# Autodesk Inventor assembly: 42146-34
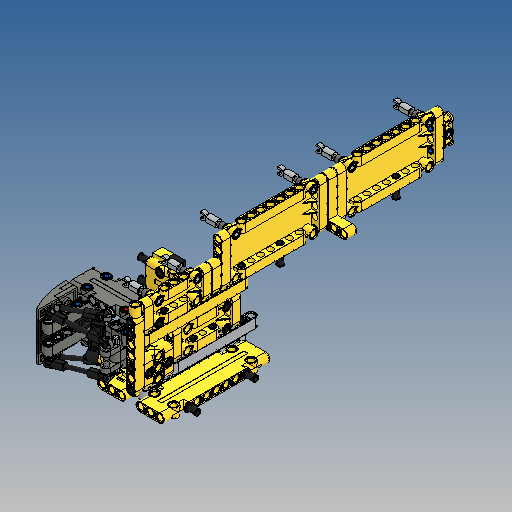
[picture p0: Inventor's stored thumbnail of the model, 512x512]
Saved by Autodesk Inventor 2025 (Build 290162010, 162A)
## iProperties
Created: 2024-12-06
Part Number: 42146-34
Material: Generisch
Document SubType Name: Assembly
Designer: hp.muther
Author: hp.muther
## Documents named in this file (48)
- D:\Inventor\Projekte\Muther\LEGO Technic\LEGO Technik - Raupenkran LR 13000 (42146)\42146-34.iam
- D:\Inventor\Projekte\Muther\LEGO Technic\LEGO Pieces\Paneelen\18945-Yellow.ipt
- D:\Inventor\Projekte\Muther\LEGO Technic\LEGO Pieces\Lochbalken\73507-LtBluishGray.ipt
- D:\Inventor\Projekte\Muther\LEGO Technic\LEGO Pieces\Paneelen\15458-Yellow.ipt
- D:\Inventor\Projekte\Muther\LEGO Technic\LEGO Pieces\Pin's\6558-Blue.ipt
- D:\Inventor\Projekte\Muther\LEGO Technic\LEGO Pieces\Pin's\2780-Black.ipt
- D:\Inventor\Projekte\Muther\LEGO Technic\LEGO Pieces\Pin's\32054-LtBluishGray.ipt
- D:\Inventor\Projekte\Muther\LEGO Technic\LEGO Pieces\Pin's\43093-Blue.ipt
- D:\Inventor\Projekte\Muther\LEGO Technic\LEGO Pieces\Pin's\4274-LtBluishGray.ipt
- D:\Inventor\Projekte\Muther\LEGO Technic\LEGO Pieces\Verbindungselemente\32184-Yellow.ipt
- D:\Inventor\Projekte\Muther\LEGO Technic\LEGO Pieces\Verbindungselemente\39793-Yellow.ipt
- D:\Inventor\Projekte\Muther\LEGO Technic\LEGO Pieces\Winkel\32526-Yellow.ipt
- D:\Inventor\Projekte\Muther\LEGO Technic\LEGO Pieces\Lochbalken\32523-Yellow.ipt
- D:\Inventor\Projekte\Muther\LEGO Technic\LEGO Pieces\Lochbalken\32525-Yellow.ipt
- D:\Inventor\Projekte\Muther\LEGO Technic\LEGO Pieces\Lochbalken\32524-Yellow.ipt
- D:\Inventor\Projekte\Muther\LEGO Technic\LEGO Pieces\Lochbalken\40490-LtBluishGray.ipt
- D:\Inventor\Projekte\Muther\LEGO Technic\LEGO Pieces\Paneelen\64782-Yellow.ipt
- D:\Inventor\Projekte\Muther\LEGO Technic\LEGO Pieces\Paneelen\71709-Yellow.ipt
- D:\Inventor\Projekte\Muther\LEGO Technic\LEGO Pieces\Verbindungselemente\15100-Yellow.ipt
- D:\Inventor\Projekte\Muther\LEGO Technic\LEGO Pieces\Achsen\78258-DarkStoneGrey.ipt
- D:\Inventor\Projekte\Muther\LEGO Technic\LEGO Pieces\Diverses\44873-LtBluishGray.ipt
- D:\Inventor\Projekte\Muther\LEGO Technic\LEGO Pieces\Steine\32000-Black.ipt
- D:\Inventor\Projekte\Muther\LEGO Technic\LEGO Pieces\Steine\3894-Yellow.ipt
- D:\Inventor\Projekte\Muther\LEGO Technic\LEGO Pieces\Lochbalken\32524-DkBluishGray.ipt
- D:\Inventor\Projekte\Muther\LEGO Technic\LEGO Pieces\Rund\18654-DkBluishGray.ipt
- D:\Inventor\Projekte\Muther\LEGO Technic\LEGO Pieces\Winkel\32140-DkBluishGray.ipt
- D:\Inventor\Projekte\Muther\LEGO Technic\LEGO Pieces\Paneelen\71709-DkBluishGray.ipt
- D:\Inventor\Projekte\Muther\LEGO Technic\LEGO Pieces\Winkel\32056-DkBluishGray.ipt
- D:\Inventor\Projekte\Muther\LEGO Technic\LEGO Pieces\Pin's\11214-Red.ipt
- D:\Inventor\Projekte\Muther\LEGO Technic\LEGO Pieces\Platten, Kacheln\18677-Black.ipt
- D:\Inventor\Projekte\Muther\LEGO Technic\LEGO Technik - Raupenkran LR 13000 (42146)\42146_63864_1.ipt
- D:\Inventor\Projekte\Muther\LEGO Technic\LEGO Pieces\Lochbalken\60483-DkBluishGray.ipt
- D:\Inventor\Projekte\Muther\LEGO Technic\LEGO Pieces\Lochbalken schmal\41677-DKBluishGray.ipt
- D:\Inventor\Projekte\Muther\LEGO Technic\LEGO Pieces\Achsen\4519-LtBluishGray.ipt
- D:\Inventor\Projekte\Muther\LEGO Technic\LEGO Pieces\Diverses\48729-DkBluishGray.ipt
- D:\Inventor\Projekte\Muther\LEGO Technic\LEGO Pieces\Achsen\87994-Black.ipt
- D:\Inventor\Projekte\Muther\LEGO Technic\LEGO Pieces\Diverses\23443-Black.ipt
- D:\Inventor\Projekte\Muther\LEGO Technic\LEGO Pieces\Steine rund\98138-TransOrange.ipt
- D:\Inventor\Projekte\Muther\LEGO Technic\LEGO Pieces\Platten, Kacheln\63864-DkBluishGray.ipt
- D:\Inventor\Projekte\Muther\LEGO Technic\LEGO Pieces\Platten, Kacheln\3623-DkBluishGray.ipt
- D:\Inventor\Projekte\Muther\LEGO Technic\LEGO Pieces\Platten, Kacheln\3021-DkBluishGray.ipt
- D:\Inventor\Projekte\Muther\LEGO Technic\LEGO Pieces\Platten, Kacheln\3022-DkBluishGray.ipt
- D:\Inventor\Projekte\Muther\LEGO Technic\LEGO Pieces\Steine schräg\11153-Black.ipt
- D:\Inventor\Projekte\Muther\LEGO Technic\LEGO Pieces\Platten, Kacheln\11212-DkBluishGray.ipt
- D:\Inventor\Projekte\Muther\LEGO Technic\LEGO Pieces\Steine schräg\11153-DkBluishGray.ipt
- D:\Inventor\Projekte\Muther\LEGO Technic\LEGO Pieces\Platten, Kacheln\3070-DkBluishGray.ipt
- D:\Inventor\Projekte\Muther\LEGO Technic\LEGO Pieces\Platten, Kacheln\3024-DkBluishGray.ipt
- D:\Inventor\Projekte\Muther\LEGO Technic\LEGO Pieces\Platten, Kacheln\93606-Black.ipt
## Components (147 placed, 47 different names)
1. 18945-Yellow:1 — Einfügen:1, Einfügen:6, Passend:2
2. 73507-LtBluishGray:1 — Einfügen:2, Einfügen:3, Einfügen:6, Einfügen:7, Einfügen:45, Passend:12
3. 15458-Yellow:1 — Einfügen:4, Einfügen:5, Einfügen:7, Passend:1
4. 6558-Blue:1 — Einfügen:2
5. 6558-Blue:2 — Einfügen:3, Passend:1, Passend:2
6. 2780-Black:1 — Einfügen:4
7. 32054-LtBluishGray:1 — Einfügen:1
8. 2780-Black:2 — Einfügen:5
9. 43093-Blue:1 — Einfügen:8
10. 43093-Blue:2 — Einfügen:9, Passend:3
11. 6558-Blue:3 — Einfügen:11, Passend:4, Passend:5
12. 6558-Blue:4 — Einfügen:12
13. 2780-Black:3 — Einfügen:15, Passend:8
14. 6558-Blue:5 — Einfügen:16
15. 6558-Blue:6 — Einfügen:17, Passend:6, Passend:7
16. 2780-Black:4 — Einfügen:21
17. 2780-Black:5 — Einfügen:20
18. 2780-Black:6 — Einfügen:19
19. 2780-Black:7 — Einfügen:30
20. 2780-Black:8 — Einfügen:31, Passend:11
21. 2780-Black:9 — Einfügen:26, Passend:10
22. 2780-Black:12 — Einfügen:27, Passend:9
23. 2780-Black:13 — Einfügen:28
24. 2780-Black:14 — Einfügen:34, Passend:12
25. 2780-Black:15 — Einfügen:35
26. 2780-Black:16 — Einfügen:36
27. 2780-Black:17 — Einfügen:37
28. 4274-LtBluishGray:1 — Einfügen:46, Einfügen:48
29. 2780-Black:18 — Einfügen:40, Passend:78
30. 2780-Black:19 — Einfügen:41
31. 2780-Black:20 — Einfügen:42
32. 2780-Black:21 — Einfügen:43, Passend:21
33. 2780-Black:22 — Einfügen:44, Passend:79
34. 32184-Yellow:1 — Einfügen:8, Einfügen:9, Einfügen:10, Einfügen:66
35. 39793-Yellow:1 — Einfügen:30, Einfügen:31, Einfügen:32, Fluchtend:1, Einfügen:40, Einfügen:41, Passend:77
36. 32526-Yellow:1 — Einfügen:11, Einfügen:12, Einfügen:13, Einfügen:14
37. 32523-Yellow:1 — Einfügen:16, Einfügen:17, Einfügen:18, Einfügen:22
38. 32525-Yellow:1 — Einfügen:23, Passend:8, Einfügen:29, Passend:9
39. 32524-Yellow:1 — Einfügen:39, Passend:11
40. 40490-LtBluishGray:1 — Einfügen:33, Passend:10, Einfügen:34, Einfügen:35, Einfügen:45
41. 64782-Yellow:1 — Einfügen:10, Passend:3, Einfügen:13, Passend:4, Einfügen:37, Einfügen:64, Einfügen:65
42. 71709-Yellow:1 — Einfügen:19, Einfügen:20, Einfügen:21, Einfügen:22, Passend:7, Einfügen:23, Einfügen:38, Fluchtend:2, Einfügen:39, Einfügen:44, Einfügen:46, Einfügen:61
43. 15100-Yellow:1 — Einfügen:38, Fluchtend:2
44. 64782-Yellow:2 — Einfügen:14, Passend:5, Einfügen:18, Passend:6, Einfügen:15, Einfügen:36, Einfügen:62, Einfügen:63
45. 2780-Black:23
46. 2780-Black:24
47. 71709-Yellow:2 — Einfügen:26, Einfügen:27, Einfügen:28, Einfügen:29, Einfügen:32, Fluchtend:1, Einfügen:33, Einfügen:42, Einfügen:43, Einfügen:72
48. 44873-LtBluishGray:1 — Einfügen:47, Passend:13
49. 78258-DarkStoneGrey:1 — Einfügen:47, Einfügen:48
50. 4274-LtBluishGray:2 — Einfügen:61
51. 44873-LtBluishGray:2 — Passend:13
52. 78258-DarkStoneGrey:2
53. 4274-LtBluishGray:3 — Einfügen:62
54. 44873-LtBluishGray:3 — Passend:14
55. 78258-DarkStoneGrey:3
56. 4274-LtBluishGray:4 — Einfügen:63
57. 44873-LtBluishGray:4 — Passend:14, Passend:15
58. 78258-DarkStoneGrey:4
59. 4274-LtBluishGray:5 — Einfügen:66
60. 44873-LtBluishGray:5 — Winkel:1
61. 78258-DarkStoneGrey:5
62. 4274-LtBluishGray:6 — Einfügen:65
63. 44873-LtBluishGray:6 — Passend:16, Winkel:1
64. 78258-DarkStoneGrey:6
65. 4274-LtBluishGray:7 — Einfügen:64
66. 44873-LtBluishGray:7 — Passend:15, Passend:16
67. 78258-DarkStoneGrey:7
68. 2780-Black:25 — Einfügen:67, Passend:20
69. 2780-Black:26 — Einfügen:68
70. 71709-Yellow:3 — Einfügen:67, Einfügen:68, Einfügen:69, Einfügen:70, Einfügen:71, Einfügen:72, Passend:21
71. 2780-Black:27 — Einfügen:70
72. 2780-Black:28 — Einfügen:69
73. 32000-Black:1 — Passend:18, Fluchtend:5, Passend:19, Passend:20
74. 32000-Black:2 — Passend:17, Fluchtend:3, Fluchtend:4, Passend:19, Einfügen:71
75. 3894-Yellow:1 — Passend:17, Passend:18, Fluchtend:3, Fluchtend:4, Fluchtend:5
76. 32524-DkBluishGray:1 — Einfügen:73, Einfügen:74, Einfügen:77, Einfügen:78, Einfügen:79, Einfügen:80, Einfügen:81, Einfügen:82, Einfügen:85
77. 32000-Black:3 — Einfügen:81, Passend:75
78. 32000-Black:4 — Einfügen:82, Einfügen:83, Fluchtend:18
79. 4274-LtBluishGray:8 — Einfügen:73, Einfügen:108
80. 4274-LtBluishGray:9 — Einfügen:74, Einfügen:109
81. 6558-Blue:7 — Einfügen:77
82. 6558-Blue:8 — Einfügen:80, Passend:24
83. 6558-Blue:9 — Einfügen:79, Passend:23
84. 6558-Blue:10 — Einfügen:78
85. 32524-DkBluishGray:2 — Einfügen:83, Passend:23, Einfügen:103, Einfügen:104, Einfügen:107
86. 4274-LtBluishGray:10 — Einfügen:111
87. 4274-LtBluishGray:11 — Einfügen:110
88. 4274-LtBluishGray:12 — Einfügen:84, Einfügen:113
89. 6558-Blue:11 — Einfügen:87, Passend:31
90. 43093-Blue:3 — Einfügen:86, Einfügen:88
91. 18654-DkBluishGray:1 — Einfügen:89
92. 32140-DkBluishGray:1 — Einfügen:88, Passend:25, Einfügen:89, Einfügen:87, Einfügen:93, Passend:27, Einfügen:100
93. 71709-DkBluishGray:1 — Einfügen:84, Einfügen:85, Passend:24, Einfügen:86, Passend:25, Passend:76, Passend:79
94. 32056-DkBluishGray:1 — Einfügen:90, Passend:26, Einfügen:92, Einfügen:94, Winkel:2, Winkel:3
95. 32056-DkBluishGray:2 — Einfügen:90, Passend:26, Einfügen:91, Passend:27
96. 43093-Blue:4 — Einfügen:92
97. 11214-Red:1 — Einfügen:91, Einfügen:93
98. 15100-Yellow:2 — Einfügen:94, Einfügen:95, Winkel:2
99. 18677-Black:1 — Passend:28, Fluchtend:6, Fluchtend:7, Einfügen:95
100. 42146_63864_1:1 — Passend:28, Fluchtend:6, Fluchtend:7
101. 6558-Blue:12 — Einfügen:99
102. 60483-DkBluishGray:1 — Einfügen:96, Einfügen:97, Einfügen:98, Einfügen:99, Einfügen:100, Winkel:3, Einfügen:101
103. 41677-DKBluishGray:1 — Einfügen:97, Passend:29, Einfügen:114
104. 41677-DKBluishGray:2 — Einfügen:98, Passend:30, Einfügen:115
105. 4519-LtBluishGray:1 — Einfügen:96, Passend:29, Passend:30
106. 32140-DkBluishGray:2 — Einfügen:101, Passend:31, Einfügen:102, Einfügen:106
107. 43093-Blue:5 — Einfügen:102
108. 2780-Black:29 — Einfügen:103
109. 2780-Black:30 — Einfügen:104
110. 71709-DkBluishGray:2 — Einfügen:105, Einfügen:107, Passend:32, Passend:77, Passend:78
111. 4274-LtBluishGray:13 — Einfügen:105, Einfügen:112
112. 2780-Black:31 — Einfügen:106, Passend:32
113. 48729-DkBluishGray:1 — Einfügen:108, Passend:35, Passend:36
114. 48729-DkBluishGray:2 — Einfügen:109, Einfügen:125
115. 48729-DkBluishGray:3 — Einfügen:113, Einfügen:120
116. 48729-DkBluishGray:4 — Einfügen:115, Einfügen:123
117. 48729-DkBluishGray:5 — Einfügen:110, Einfügen:124
118. 48729-DkBluishGray:6 — Einfügen:112, Einfügen:121
119. 48729-DkBluishGray:7 — Einfügen:111, Passend:37, Passend:38
120. 48729-DkBluishGray:8 — Einfügen:114, Einfügen:122
121. 87994-Black:1 — Einfügen:116, Passend:35, Passend:36
122. 23443-Black:1 — Einfügen:116, Einfügen:120
123. 87994-Black:2 — Passend:33
124. 23443-Black:2 — Einfügen:122
125. 23443-Black:3 — Passend:33, Einfügen:125
126. 87994-Black:3
127. 23443-Black:4 — Einfügen:123
128. 23443-Black:5 — Einfügen:124
129. 87994-Black:4 — Passend:37, Passend:38
130. 23443-Black:6 — Einfügen:121
131. 98138-TransOrange:1 — Einfügen:126
132. 63864-DkBluishGray:1 — Passend:47, Fluchtend:12, Fluchtend:13, Passend:49, Passend:53, Passend:54, Fluchtend:14, Passend:67, Passend:71, Passend:72
133. 63864-DkBluishGray:2 — Passend:57, Passend:58, Fluchtend:15, Passend:73
134. 3623-DkBluishGray:1 — Passend:39, Fluchtend:8, Fluchtend:9, Passend:41, Fluchtend:13
135. 3021-DkBluishGray:1 — Passend:42, Passend:43, Passend:45, Fluchtend:11, Passend:46, Passend:59
136. 3022-DkBluishGray:1 — Passend:44, Passend:45, Fluchtend:11, Passend:60
137. 11153-Black:1 — Passend:64, Passend:69, Passend:70, Passend:73
138. 11212-DkBluishGray:1 — Passend:39, Fluchtend:8, Fluchtend:9, Passend:40, Fluchtend:10, Passend:43, Passend:46, Passend:75, Passend:76, Fluchtend:18
139. 11153-DkBluishGray:1 — Passend:65, Passend:70, Passend:74
140. 11153-DkBluishGray:2 — Passend:66, Passend:67, Passend:68, Passend:71
141. 3070-DkBluishGray:1 — Passend:52, Passend:53, Passend:55, Passend:58, Fluchtend:15
142. 3070-DkBluishGray:2 — Passend:50, Passend:51, Passend:54, Passend:56, Fluchtend:14
143. 3024-DkBluishGray:1 — Passend:48, Passend:49, Passend:55, Passend:56, Einfügen:126
144. 93606-Black:1 — Passend:63, Passend:68, Passend:69, Passend:72
145. 11212-DkBluishGray:2 — Passend:40, Passend:41, Fluchtend:10, Passend:47, Fluchtend:12, Passend:48, Passend:50, Passend:42, Passend:51, Passend:52, Passend:57, Passend:61, Passend:62, Fluchtend:16, Fluchtend:17, Passend:44, Passend:63, Passend:64
146. 3024-DkBluishGray:2 — Passend:59, Passend:62, Fluchtend:16, Passend:66
147. 3024-DkBluishGray:3 — Passend:60, Passend:61, Fluchtend:17, Passend:65, Passend:74
## Relationships (226: Insert 126, Mate 79, Flush 18, Angle 3)
- Winkel:2 [Angle] (20 deg): 32056-DkBluishGray:1 ↔ 15100-Yellow:2
- Einfügen:1 [Insert]: 18945-Yellow:1 ↔ 32054-LtBluishGray:1
- Einfügen:2 [Insert]: 73507-LtBluishGray:1 ↔ 6558-Blue:1
- Einfügen:3 [Insert]: 73507-LtBluishGray:1 ↔ 6558-Blue:2
- Einfügen:4 [Insert]: 15458-Yellow:1 ↔ 2780-Black:1
- Einfügen:5 [Insert]: 15458-Yellow:1 ↔ 2780-Black:2
- Einfügen:6 [Insert]: 18945-Yellow:1 ↔ 73507-LtBluishGray:1
- Einfügen:7 [Insert]: 73507-LtBluishGray:1 ↔ 15458-Yellow:1
- Passend:1 [Mate]: 15458-Yellow:1 ↔ 6558-Blue:2
- Passend:2 [Mate]: 18945-Yellow:1 ↔ 6558-Blue:2
- Einfügen:8 [Insert]: 43093-Blue:1 ↔ 32184-Yellow:1
- Einfügen:9 [Insert]: 43093-Blue:2 ↔ 32184-Yellow:1
- Einfügen:10 [Insert]: 32184-Yellow:1 ↔ 64782-Yellow:1
- Passend:3 [Mate]: 43093-Blue:2 ↔ 64782-Yellow:1
- Einfügen:11 [Insert]: 6558-Blue:3 ↔ 32526-Yellow:1
- Einfügen:12 [Insert]: 6558-Blue:4 ↔ 32526-Yellow:1
- Einfügen:13 [Insert]: 32526-Yellow:1 ↔ 64782-Yellow:1
- Passend:4 [Mate]: 6558-Blue:3 ↔ 64782-Yellow:1
- Einfügen:14 [Insert]: 32526-Yellow:1 ↔ 64782-Yellow:2
- Passend:5 [Mate]: 6558-Blue:3 ↔ 64782-Yellow:2
- Einfügen:15 [Insert]: 2780-Black:3 ↔ 64782-Yellow:2
- Einfügen:16 [Insert]: 6558-Blue:5 ↔ 32523-Yellow:1
- Einfügen:17 [Insert]: 6558-Blue:6 ↔ 32523-Yellow:1
- Einfügen:18 [Insert]: 32523-Yellow:1 ↔ 64782-Yellow:2
- Passend:6 [Mate]: 6558-Blue:6 ↔ 64782-Yellow:2
- Einfügen:19 [Insert]: 2780-Black:6 ↔ 71709-Yellow:1
- Einfügen:20 [Insert]: 2780-Black:5 ↔ 71709-Yellow:1
- Einfügen:21 [Insert]: 2780-Black:4 ↔ 71709-Yellow:1
- Einfügen:22 [Insert]: 32523-Yellow:1 ↔ 71709-Yellow:1
- Passend:7 [Mate]: 6558-Blue:6 ↔ 71709-Yellow:1
- Einfügen:23 [Insert]: 32525-Yellow:1 ↔ 71709-Yellow:1
- Passend:8 [Mate]: 2780-Black:3 ↔ 32525-Yellow:1
- [Insert]: 2780-Black:24 ↔ 71709-Yellow:2
- [Insert]: 2780-Black:23 ↔ 71709-Yellow:2
- Einfügen:26 [Insert]: 2780-Black:9 ↔ 71709-Yellow:2
- Einfügen:27 [Insert]: 2780-Black:12 ↔ 71709-Yellow:2
- Einfügen:28 [Insert]: 2780-Black:13 ↔ 71709-Yellow:2
- Einfügen:29 [Insert]: 32525-Yellow:1 ↔ 71709-Yellow:2
- Passend:9 [Mate]: 2780-Black:12 ↔ 32525-Yellow:1
- Einfügen:30 [Insert]: 2780-Black:7 ↔ 39793-Yellow:1
- Einfügen:31 [Insert]: 2780-Black:8 ↔ 39793-Yellow:1
- Einfügen:32 [Insert]: 39793-Yellow:1 ↔ 71709-Yellow:2
- Fluchtend:1 [Flush]: 39793-Yellow:1 ↔ 71709-Yellow:2
- Einfügen:33 [Insert]: 40490-LtBluishGray:1 ↔ 71709-Yellow:2
- Passend:10 [Mate]: 2780-Black:9 ↔ 40490-LtBluishGray:1
- Einfügen:34 [Insert]: 2780-Black:14 ↔ 40490-LtBluishGray:1
- Einfügen:35 [Insert]: 2780-Black:15 ↔ 40490-LtBluishGray:1
- Einfügen:36 [Insert]: 2780-Black:16 ↔ 64782-Yellow:2
- Einfügen:37 [Insert]: 2780-Black:17 ↔ 64782-Yellow:1
- Einfügen:38 [Insert]: 71709-Yellow:1 ↔ 15100-Yellow:1
- Fluchtend:2 [Flush]: 71709-Yellow:1 ↔ 15100-Yellow:1
- Einfügen:39 [Insert]: 32524-Yellow:1 ↔ 71709-Yellow:1
- Passend:11 [Mate]: 2780-Black:8 ↔ 32524-Yellow:1
- Einfügen:40 [Insert]: 2780-Black:18 ↔ 39793-Yellow:1
- Einfügen:41 [Insert]: 2780-Black:19 ↔ 39793-Yellow:1
- Einfügen:42 [Insert]: 2780-Black:20 ↔ 71709-Yellow:2
- Einfügen:43 [Insert]: 2780-Black:21 ↔ 71709-Yellow:2
- Einfügen:44 [Insert]: 2780-Black:22 ↔ 71709-Yellow:1
- Einfügen:45 [Insert]: 73507-LtBluishGray:1 ↔ 40490-LtBluishGray:1
- Passend:12 [Mate]: 73507-LtBluishGray:1 ↔ 2780-Black:14
- Einfügen:46 [Insert]: 4274-LtBluishGray:1 ↔ 71709-Yellow:1
- Einfügen:47 [Insert]: 44873-LtBluishGray:1 ↔ 78258-DarkStoneGrey:1
- Einfügen:48 [Insert]: 4274-LtBluishGray:1 ↔ 78258-DarkStoneGrey:1
- [Insert]: 44873-LtBluishGray:2 ↔ 78258-DarkStoneGrey:2
- [Insert]: 4274-LtBluishGray:2 ↔ 78258-DarkStoneGrey:2
- [Insert]: 44873-LtBluishGray:3 ↔ 78258-DarkStoneGrey:3
- [Insert]: 4274-LtBluishGray:3 ↔ 78258-DarkStoneGrey:3
- [Insert]: 44873-LtBluishGray:4 ↔ 78258-DarkStoneGrey:4
- [Insert]: 4274-LtBluishGray:4 ↔ 78258-DarkStoneGrey:4
- [Insert]: 44873-LtBluishGray:5 ↔ 78258-DarkStoneGrey:5
- [Insert]: 4274-LtBluishGray:5 ↔ 78258-DarkStoneGrey:5
- [Insert]: 44873-LtBluishGray:6 ↔ 78258-DarkStoneGrey:6
- [Insert]: 4274-LtBluishGray:6 ↔ 78258-DarkStoneGrey:6
- [Insert]: 44873-LtBluishGray:7 ↔ 78258-DarkStoneGrey:7
- [Insert]: 4274-LtBluishGray:7 ↔ 78258-DarkStoneGrey:7
- Einfügen:61 [Insert]: 71709-Yellow:1 ↔ 4274-LtBluishGray:2
- Einfügen:62 [Insert]: 64782-Yellow:2 ↔ 4274-LtBluishGray:3
- Einfügen:63 [Insert]: 64782-Yellow:2 ↔ 4274-LtBluishGray:4
- Einfügen:64 [Insert]: 64782-Yellow:1 ↔ 4274-LtBluishGray:7
- Einfügen:65 [Insert]: 64782-Yellow:1 ↔ 4274-LtBluishGray:6
- Einfügen:66 [Insert]: 32184-Yellow:1 ↔ 4274-LtBluishGray:5
- Passend:13 [Mate]: 44873-LtBluishGray:1 ↔ 44873-LtBluishGray:2
- Passend:14 [Mate]: 44873-LtBluishGray:3 ↔ 44873-LtBluishGray:4
- Passend:15 [Mate]: 44873-LtBluishGray:4 ↔ 44873-LtBluishGray:7
- Passend:16 [Mate]: 44873-LtBluishGray:6 ↔ 44873-LtBluishGray:7
- Winkel:1 [Angle] (90 deg): 44873-LtBluishGray:5 ↔ 44873-LtBluishGray:6
- Einfügen:67 [Insert]: 2780-Black:25 ↔ 71709-Yellow:3
- Einfügen:68 [Insert]: 2780-Black:26 ↔ 71709-Yellow:3
- Einfügen:69 [Insert]: 71709-Yellow:3 ↔ 2780-Black:28
- Einfügen:70 [Insert]: 71709-Yellow:3 ↔ 2780-Black:27
- Passend:17 [Mate]: 32000-Black:2 ↔ 3894-Yellow:1
- Passend:18 [Mate]: 32000-Black:1 ↔ 3894-Yellow:1
- Fluchtend:3 [Flush]: 32000-Black:2 ↔ 3894-Yellow:1
- Fluchtend:4 [Flush]: 32000-Black:2 ↔ 3894-Yellow:1
- Fluchtend:5 [Flush]: 32000-Black:1 ↔ 3894-Yellow:1
- Passend:19 [Mate]: 32000-Black:1 ↔ 32000-Black:2
- Einfügen:71 [Insert]: 71709-Yellow:3 ↔ 32000-Black:2
- Passend:20 [Mate]: 2780-Black:25 ↔ 32000-Black:1
- Einfügen:72 [Insert]: 71709-Yellow:2 ↔ 71709-Yellow:3
- Passend:21 [Mate]: 2780-Black:21 ↔ 71709-Yellow:3
- [Mate]: 32000-Black:3 ↔ 32000-Black:4
- Einfügen:73 [Insert]: 32524-DkBluishGray:1 ↔ 4274-LtBluishGray:8
- Einfügen:74 [Insert]: 32524-DkBluishGray:1 ↔ 4274-LtBluishGray:9
- [Insert]: 32524-DkBluishGray:2 ↔ 4274-LtBluishGray:10
- [Insert]: 32524-DkBluishGray:2 ↔ 4274-LtBluishGray:11
- Einfügen:77 [Insert]: 32524-DkBluishGray:1 ↔ 6558-Blue:7
- Einfügen:78 [Insert]: 32524-DkBluishGray:1 ↔ 6558-Blue:10
- Einfügen:79 [Insert]: 32524-DkBluishGray:1 ↔ 6558-Blue:9
- Einfügen:80 [Insert]: 32524-DkBluishGray:1 ↔ 6558-Blue:8
- Einfügen:81 [Insert]: 32524-DkBluishGray:1 ↔ 32000-Black:3
- Einfügen:82 [Insert]: 32524-DkBluishGray:1 ↔ 32000-Black:4
- Einfügen:83 [Insert]: 32000-Black:4 ↔ 32524-DkBluishGray:2
- Passend:23 [Mate]: 6558-Blue:9 ↔ 32524-DkBluishGray:2
- Einfügen:84 [Insert]: 4274-LtBluishGray:12 ↔ 71709-DkBluishGray:1
- Einfügen:85 [Insert]: 32524-DkBluishGray:1 ↔ 71709-DkBluishGray:1
- Passend:24 [Mate]: 6558-Blue:8 ↔ 71709-DkBluishGray:1
- Einfügen:86 [Insert]: 43093-Blue:3 ↔ 71709-DkBluishGray:1
- Einfügen:87 [Insert]: 6558-Blue:11 ↔ 32140-DkBluishGray:1
- Einfügen:88 [Insert]: 43093-Blue:3 ↔ 32140-DkBluishGray:1
- Passend:25 [Mate]: 32140-DkBluishGray:1 ↔ 71709-DkBluishGray:1
- Einfügen:89 [Insert]: 18654-DkBluishGray:1 ↔ 32140-DkBluishGray:1
- Einfügen:90 [Insert]: 32056-DkBluishGray:1 ↔ 32056-DkBluishGray:2
- Passend:26 [Mate]: 32056-DkBluishGray:1 ↔ 32056-DkBluishGray:2
- Einfügen:91 [Insert]: 32056-DkBluishGray:2 ↔ 11214-Red:1
- Einfügen:92 [Insert]: 32056-DkBluishGray:1 ↔ 43093-Blue:4
- Einfügen:93 [Insert]: 32140-DkBluishGray:1 ↔ 11214-Red:1
- Passend:27 [Mate]: 32140-DkBluishGray:1 ↔ 32056-DkBluishGray:2
- Einfügen:94 [Insert]: 32056-DkBluishGray:1 ↔ 15100-Yellow:2
- Passend:28 [Mate]: 18677-Black:1 ↔ 42146_63864_1:1
- Fluchtend:6 [Flush]: 18677-Black:1 ↔ 42146_63864_1:1
- Fluchtend:7 [Flush]: 18677-Black:1 ↔ 42146_63864_1:1
- Einfügen:95 [Insert]: 15100-Yellow:2 ↔ 18677-Black:1
- Einfügen:96 [Insert] (-16 mm): 60483-DkBluishGray:1 ↔ 4519-LtBluishGray:1
- Einfügen:97 [Insert]: 60483-DkBluishGray:1 ↔ 41677-DKBluishGray:1
- Einfügen:98 [Insert]: 60483-DkBluishGray:1 ↔ 41677-DKBluishGray:2
- Passend:29 [Mate]: 41677-DKBluishGray:1 ↔ 4519-LtBluishGray:1
- Passend:30 [Mate]: 41677-DKBluishGray:2 ↔ 4519-LtBluishGray:1
- Einfügen:99 [Insert]: 6558-Blue:12 ↔ 60483-DkBluishGray:1
- Einfügen:100 [Insert]: 32140-DkBluishGray:1 ↔ 60483-DkBluishGray:1
- Winkel:3 [Angle] (0 deg): 32056-DkBluishGray:1 ↔ 60483-DkBluishGray:1
- Einfügen:101 [Insert]: 60483-DkBluishGray:1 ↔ 32140-DkBluishGray:2
- Passend:31 [Mate]: 6558-Blue:11 ↔ 32140-DkBluishGray:2
- Einfügen:102 [Insert]: 32140-DkBluishGray:2 ↔ 43093-Blue:5
- Einfügen:103 [Insert]: 32524-DkBluishGray:2 ↔ 2780-Black:29
- Einfügen:104 [Insert]: 32524-DkBluishGray:2 ↔ 2780-Black:30
- Einfügen:105 [Insert]: 71709-DkBluishGray:2 ↔ 4274-LtBluishGray:13
- Einfügen:106 [Insert]: 32140-DkBluishGray:2 ↔ 2780-Black:31
- Einfügen:107 [Insert]: 32524-DkBluishGray:2 ↔ 71709-DkBluishGray:2
- Passend:32 [Mate]: 71709-DkBluishGray:2 ↔ 2780-Black:31
- Einfügen:108 [Insert] (-8 mm): 4274-LtBluishGray:8 ↔ 48729-DkBluishGray:1
- Einfügen:109 [Insert] (-8 mm): 4274-LtBluishGray:9 ↔ 48729-DkBluishGray:2
- Einfügen:110 [Insert] (-8 mm): 4274-LtBluishGray:11 ↔ 48729-DkBluishGray:5
- Einfügen:111 [Insert] (-8 mm): 4274-LtBluishGray:10 ↔ 48729-DkBluishGray:7
- Einfügen:112 [Insert] (-8 mm): 4274-LtBluishGray:13 ↔ 48729-DkBluishGray:6
- Einfügen:113 [Insert] (-8 mm): 4274-LtBluishGray:12 ↔ 48729-DkBluishGray:3
- Einfügen:114 [Insert] (-8 mm): 41677-DKBluishGray:1 ↔ 48729-DkBluishGray:8
- Einfügen:115 [Insert] (-8 mm): 41677-DKBluishGray:2 ↔ 48729-DkBluishGray:4
- Einfügen:116 [Insert]: 87994-Black:1 ↔ 23443-Black:1
- [Insert]: 87994-Black:2 ↔ 23443-Black:2
- Passend:33 [Mate]: 87994-Black:2 ↔ 23443-Black:3
- [Insert]: 87994-Black:3 ↔ 23443-Black:4
- [Mate]: 87994-Black:3 ↔ 23443-Black:5
- [Insert]: 87994-Black:4 ↔ 23443-Black:6
- Einfügen:120 [Insert]: 48729-DkBluishGray:3 ↔ 23443-Black:1
- Passend:35 [Mate]: 48729-DkBluishGray:1 ↔ 87994-Black:1
- Passend:36 [Mate]: 48729-DkBluishGray:1 ↔ 87994-Black:1
- Einfügen:121 [Insert]: 48729-DkBluishGray:6 ↔ 23443-Black:6
- Passend:37 [Mate]: 48729-DkBluishGray:7 ↔ 87994-Black:4
- Passend:38 [Mate]: 48729-DkBluishGray:7 ↔ 87994-Black:4
- Einfügen:122 [Insert]: 48729-DkBluishGray:8 ↔ 23443-Black:2
- Einfügen:123 [Insert]: 48729-DkBluishGray:4 ↔ 23443-Black:4
- Einfügen:124 [Insert]: 48729-DkBluishGray:5 ↔ 23443-Black:5
- Einfügen:125 [Insert]: 48729-DkBluishGray:2 ↔ 23443-Black:3
- Passend:39 [Mate]: 3623-DkBluishGray:1 ↔ 11212-DkBluishGray:1
- Fluchtend:8 [Flush]: 3623-DkBluishGray:1 ↔ 11212-DkBluishGray:1
- Fluchtend:9 [Flush]: 3623-DkBluishGray:1 ↔ 11212-DkBluishGray:1
- Passend:40 [Mate]: 11212-DkBluishGray:1 ↔ 11212-DkBluishGray:2
- Passend:41 [Mate]: 3623-DkBluishGray:1 ↔ 11212-DkBluishGray:2
- Fluchtend:10 [Flush]: 11212-DkBluishGray:1 ↔ 11212-DkBluishGray:2
- Passend:42 [Mate]: 3021-DkBluishGray:1 ↔ 11212-DkBluishGray:2
- Passend:43 [Mate]: 3021-DkBluishGray:1 ↔ 11212-DkBluishGray:1
- Passend:44 [Mate]: 3022-DkBluishGray:1 ↔ 11212-DkBluishGray:2
- Passend:45 [Mate]: 3021-DkBluishGray:1 ↔ 3022-DkBluishGray:1
- Fluchtend:11 [Flush]: 3021-DkBluishGray:1 ↔ 3022-DkBluishGray:1
- Passend:46 [Mate] (8 mm): 3021-DkBluishGray:1 ↔ 11212-DkBluishGray:1
- Passend:47 [Mate]: 63864-DkBluishGray:1 ↔ 11212-DkBluishGray:2
- Fluchtend:12 [Flush]: 63864-DkBluishGray:1 ↔ 11212-DkBluishGray:2
- Fluchtend:13 [Flush]: 63864-DkBluishGray:1 ↔ 3623-DkBluishGray:1
- Passend:48 [Mate]: 3024-DkBluishGray:1 ↔ 11212-DkBluishGray:2
- Passend:49 [Mate]: 63864-DkBluishGray:1 ↔ 3024-DkBluishGray:1
- Passend:50 [Mate]: 3070-DkBluishGray:2 ↔ 11212-DkBluishGray:2
- Passend:51 [Mate]: 3070-DkBluishGray:2 ↔ 11212-DkBluishGray:2
- Passend:52 [Mate]: 3070-DkBluishGray:1 ↔ 11212-DkBluishGray:2
- Passend:53 [Mate]: 63864-DkBluishGray:1 ↔ 3070-DkBluishGray:1
- Passend:54 [Mate]: 63864-DkBluishGray:1 ↔ 3070-DkBluishGray:2
- Passend:55 [Mate]: 3070-DkBluishGray:1 ↔ 3024-DkBluishGray:1
- Passend:56 [Mate]: 3070-DkBluishGray:2 ↔ 3024-DkBluishGray:1
- Fluchtend:14 [Flush]: 63864-DkBluishGray:1 ↔ 3070-DkBluishGray:2
- Passend:57 [Mate]: 63864-DkBluishGray:2 ↔ 11212-DkBluishGray:2
- Passend:58 [Mate]: 63864-DkBluishGray:2 ↔ 3070-DkBluishGray:1
- Fluchtend:15 [Flush]: 63864-DkBluishGray:2 ↔ 3070-DkBluishGray:1
- Passend:59 [Mate]: 3021-DkBluishGray:1 ↔ 3024-DkBluishGray:2
- Passend:60 [Mate]: 3022-DkBluishGray:1 ↔ 3024-DkBluishGray:3
- Passend:61 [Mate]: 11212-DkBluishGray:2 ↔ 3024-DkBluishGray:3
- Passend:62 [Mate]: 11212-DkBluishGray:2 ↔ 3024-DkBluishGray:2
- Fluchtend:16 [Flush]: 11212-DkBluishGray:2 ↔ 3024-DkBluishGray:2
- Fluchtend:17 [Flush]: 11212-DkBluishGray:2 ↔ 3024-DkBluishGray:3
- Passend:63 [Mate]: 93606-Black:1 ↔ 11212-DkBluishGray:2
- Passend:64 [Mate]: 11153-Black:1 ↔ 11212-DkBluishGray:2
- Passend:65 [Mate]: 11153-DkBluishGray:1 ↔ 3024-DkBluishGray:3
- Passend:66 [Mate]: 11153-DkBluishGray:2 ↔ 3024-DkBluishGray:2
- Passend:67 [Mate]: 63864-DkBluishGray:1 ↔ 11153-DkBluishGray:2
- Passend:68 [Mate]: 11153-DkBluishGray:2 ↔ 93606-Black:1
- Passend:69 [Mate]: 11153-Black:1 ↔ 93606-Black:1
- Passend:70 [Mate]: 11153-Black:1 ↔ 11153-DkBluishGray:1
- Passend:71 [Mate]: 63864-DkBluishGray:1 ↔ 11153-DkBluishGray:2
- Passend:72 [Mate]: 63864-DkBluishGray:1 ↔ 93606-Black:1
- Passend:73 [Mate]: 63864-DkBluishGray:2 ↔ 11153-Black:1
- Passend:74 [Mate]: 11153-DkBluishGray:1 ↔ 3024-DkBluishGray:3
- Einfügen:126 [Insert]: 98138-TransOrange:1 ↔ 3024-DkBluishGray:1
- Passend:75 [Mate]: 32000-Black:3 ↔ 11212-DkBluishGray:1
- Passend:76 [Mate] (0.4 mm): 71709-DkBluishGray:1 ↔ 11212-DkBluishGray:1
- Fluchtend:18 [Flush]: 32000-Black:4 ↔ 11212-DkBluishGray:1
- Passend:77 [Mate]: 39793-Yellow:1 ↔ 71709-DkBluishGray:2
- Passend:78 [Mate]: 2780-Black:18 ↔ 71709-DkBluishGray:2
- Passend:79 [Mate]: 2780-Black:22 ↔ 71709-DkBluishGray:1
## Named parameters: d31_d25 = 0 mm, d32_d26 = 0 mm, d62_d60 = 0 mm, d63_d61 = 0 mm, d64_d60 = 0 mm, d65_d61 = 0 mm, d66_d60 = 0 mm, d67_d61 = 0 mm, d68_d60 = 0 mm, d69_d61 = 0 mm, d70_d60 = 0 mm, d71_d61 = 0 mm, d72_d60 = 0 mm, d73_d61 = 0 mm, d85_d54 = 0 mm, d86_d55 = 0 mm, d99_d94 = 0 mm, d102_d100 = 0 mm, d103_d101 = 0 mm, d158_d157 = 0 mm, d160_d158_d157 = 0 mm, d161_d159 = 0 mm, d162_d157 = 0 mm
